# Autodesk Inventor assembly: Phone Holder Assembly
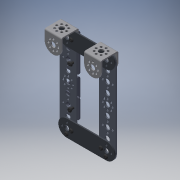
[picture p0: Inventor's stored thumbnail of the model, 180x180]
Saved by Autodesk Inventor 2016 (Build 200138000, 138)
## iProperties
Created: 2015-09-08
Part Number: Phone Holder Assembly
Document SubType Name: Assembly
Designer: phiro
Author: phiro
## Documents named in this file (6)
- C:\Users\phiro\Documents\GitHub\phi_robotics\3d-models\FTC_Tetrix_KOP_Block_Party\Tim Bloot Designs\Tutorial Bot\Phone Holder Assembly.iam
- C:\Users\phiro\Documents\GitHub\phi_robotics\3d-models\FTC_Tetrix_KOP_Block_Party\Tetrix_Kit_FTC\Autodesk Inventor Files\tetrix_739061_2012.ipt
- C:\Users\phiro\Documents\GitHub\phi_robotics\3d-models\FTC_Tetrix_KOP_Block_Party\Tetrix_Kit_FTC\Autodesk Inventor Files\tetrix_739272_2013.ipt
- C:\Users\phiro\Documents\GitHub\phi_robotics\3d-models\FTC_Tetrix_KOP_Block_Party\Tetrix_Kit_FTC\Autodesk Inventor Files\tetrix_screw-buttonhead.ipt
- C:\Users\phiro\Documents\GitHub\phi_robotics\3d-models\FTC_Tetrix_KOP_Block_Party\Tetrix_Kit_FTC\Autodesk Inventor Files\tetrix_c_channel-round.ipt
- C:\Users\phiro\Documents\GitHub\phi_robotics\3d-models\FTC_Tetrix_KOP_Block_Party\Tetrix_Kit_FTC\Autodesk Inventor Files\tetrix_inside_corner_bracket.ipt
## Components (20 placed, 5 different names)
1. tetrix_739061_2012:1 — Rigid:1, Rigid:2, Rotational:1, Rotational:2, Rotational:3, Rotational:4
2. tetrix_739061_2012:2 — Rigid:5, Rigid:6, Rotational:5, Rotational:6, Rotational:7, Rotational:8
3. tetrix_739272_2013:1 — Rigid:1, Rigid:4, Rigid:5
4. tetrix_739272_2013:2 — Rigid:2, Rigid:3, Rigid:6, Rigid:7, Rigid:8
5. tetrix_screw-buttonhead:1 — Rotational:3
6. tetrix_screw-buttonhead:2 — Rotational:4
7. tetrix_screw-buttonhead:3 — Rotational:1
8. tetrix_screw-buttonhead:4 — Rotational:2
9. tetrix_c_channel-round:1 — Rigid:3
10. tetrix_c_channel-round:2 — Rigid:4
11. tetrix_screw-buttonhead:5 — Rotational:8
12. tetrix_screw-buttonhead:6 — Rotational:7
13. tetrix_screw-buttonhead:7 — Rotational:5
14. tetrix_screw-buttonhead:8 — Rotational:6
15. tetrix_inside_corner_bracket:1 — Rigid:7
16. tetrix_inside_corner_bracket:2 — Rigid:8
17. tetrix_screw-buttonhead:9
18. tetrix_screw-buttonhead:10
19. tetrix_screw-buttonhead:11
20. tetrix_screw-buttonhead:12
## Relationships (16: WeldJoint 8, RevoluteJoint 8)
- Rigid:1 [WeldJoint]: tetrix_739061_2012:1 ↔ tetrix_739272_2013:1
- Rigid:2 [WeldJoint]: tetrix_739061_2012:1 ↔ tetrix_739272_2013:2
- Rotational:1 [RevoluteJoint]: tetrix_739061_2012:1 ↔ tetrix_screw-buttonhead:3
- Rotational:2 [RevoluteJoint]: tetrix_739061_2012:1 ↔ tetrix_screw-buttonhead:4
- Rotational:3 [RevoluteJoint]: tetrix_739061_2012:1 ↔ tetrix_screw-buttonhead:1
- Rotational:4 [RevoluteJoint]: tetrix_739061_2012:1 ↔ tetrix_screw-buttonhead:2
- Rigid:3 [WeldJoint]: tetrix_739272_2013:2 ↔ tetrix_c_channel-round:1
- Rigid:4 [WeldJoint]: tetrix_739272_2013:1 ↔ tetrix_c_channel-round:2
- Rigid:5 [WeldJoint]: tetrix_739061_2012:2 ↔ tetrix_739272_2013:1
- Rigid:6 [WeldJoint]: tetrix_739061_2012:2 ↔ tetrix_739272_2013:2
- Rotational:5 [RevoluteJoint]: tetrix_739061_2012:2 ↔ tetrix_screw-buttonhead:7
- Rotational:6 [RevoluteJoint]: tetrix_739061_2012:2 ↔ tetrix_screw-buttonhead:8
- Rotational:7 [RevoluteJoint]: tetrix_739061_2012:2 ↔ tetrix_screw-buttonhead:6
- Rotational:8 [RevoluteJoint]: tetrix_739061_2012:2 ↔ tetrix_screw-buttonhead:5
- Rigid:7 [WeldJoint]: tetrix_739272_2013:2 ↔ tetrix_inside_corner_bracket:1
- Rigid:8 [WeldJoint]: tetrix_739272_2013:2 ↔ tetrix_inside_corner_bracket:2
